# Autodesk Inventor assembly: 66-0006
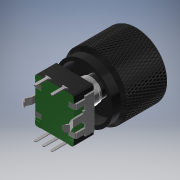
[picture p0: Inventor's stored thumbnail of the model, 180x180]
Saved by Autodesk Inventor 2018 (Build 220112000, 112)
## iProperties
Created: 2019-09-26
Part Number: 66-0006
Document SubType Name: Assembly
Designer: Bradley
Author: Bradley
## Documents named in this file (3)
- C:\Users\Bradley\Documents\GitHub\Resources\SupplierDocuments\66 - Sensor\66-0006\66-0006.iam
- C:\Users\Bradley\Documents\GitHub\Resources\SupplierDocuments\66 - Sensor\66-0006\66-0006.ipt
- C:\Users\Bradley\Documents\GitHub\Resources\SupplierDocuments\48 - Hardware\48-0076\48-0076.ipt
## Components (2 placed, 2 different names)
1. 66-0006:1 — Insert:1
2. 48-0076:1 — Insert:1
## Relationships (1: Insert 1)
- Insert:1: 66-0006:1 ↔ 48-0076:1
